# Autodesk Inventor assembly: Assembly_base_4x2
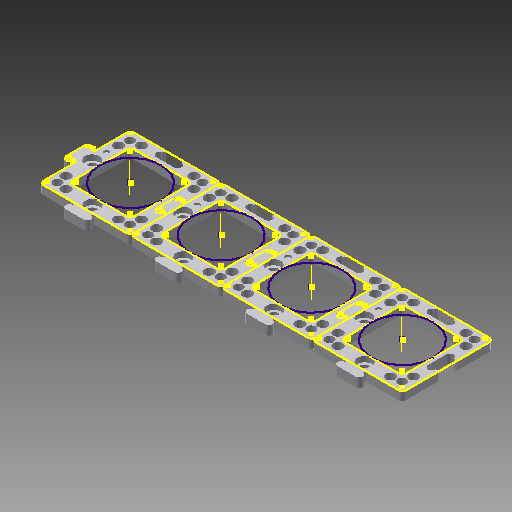
[picture p0: Inventor's stored thumbnail of the model, 512x512]
Saved by Autodesk Inventor 2019 (Build 230136000, 136)
## iProperties
Created: 2018-05-30
Part Number: Assembly_base_4x2
Material: Generisch
Document SubType Name: Assembly
Designer: diederichbenedict
Mass: 62.9957 g
Surface Area: 571.575 cm^2
Volume: 62.9957 cm^3
Density: 1 g/cm^3
Author: diederichbenedict
## Documents named in this file (2)
- C:\Users\marsikovabarbora\Dropbox\UC2\02_CAD\INVENTOR\uc2_v3\Assembly_base_4x1.iam
- C:\Users\marsikovabarbora\Dropbox\UC2\02_CAD\INVENTOR\uc2_v3\10_Base_puzzle_v3.ipt
## Components (4 placed, 1 different names)
1. 10_Base_puzzle_v3:1
2. 10_Base_puzzle_v3:2
3. 10_Base_puzzle_v3:3
4. 10_Base_puzzle_v3:4
## Component patterns: (4 elements, first: 10_Base_puzzle_v3:1)
